# Autodesk Inventor assembly: dribl-2-1
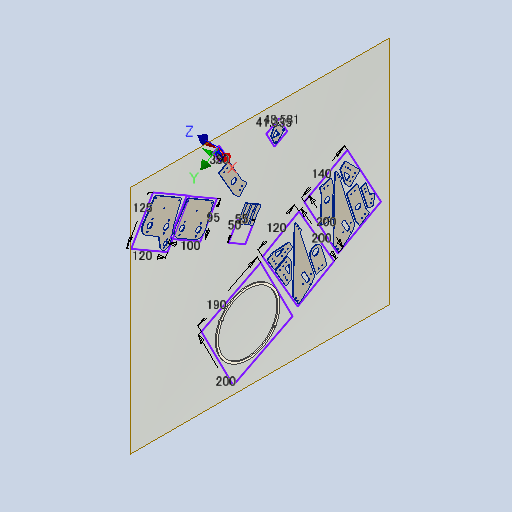
[picture p0: Inventor's stored thumbnail of the model, 512x512]
Saved by Autodesk Inventor 2025.2 (Build 292293000, 293)
## iProperties
Created: 2025-01-15
Part Number: dribl-2-1
Document SubType Name: Assembly
Designer: haruy
Author: haruy
## Documents named in this file (12)
- C:\Users\haruy\Documents\ロボコン\NHK2025\cad\cnc\dribl-2-1.iam
- C:\Users\haruy\Documents\ロボコン\NHK2025\cad\nagahisa\belt_liner\belt_liner_v2_Plate_2.ipt
- C:\Users\haruy\Documents\ロボコン\NHK2025\cad\nagahisa\dribl\dribl-v1-Plate-9.ipt
- C:\Users\haruy\Documents\ロボコン\NHK2025\cad\nagahisa\dribl\dribl-v1-Plate-6.ipt
- C:\Users\haruy\Documents\ロボコン\NHK2025\cad\nagahisa\dribl\dribl-v1-Plate-4.ipt
- C:\Users\haruy\Documents\ロボコン\NHK2025\cad\nagahisa\belt_liner\belt_liner_v2_Plate_20.ipt
- C:\Users\haruy\Documents\ロボコン\NHK2025\cad\nagahisa\dribl\dribl-v1-Plate-8.ipt
- C:\Users\haruy\Documents\ロボコン\NHK2025\cad\nagahisa\belt_liner\belt_liner_v2_Plate_19.ipt
- C:\Users\haruy\Documents\ロボコン\NHK2025\cad\nagahisa\belt_liner\belt_liner_v2_Pom_r.ipt
- C:\Users\haruy\Documents\ロボコン\NHK2025\cad\nagahisa\belt_liner\belt_liner_v4_Plate_2.ipt
- C:\Users\haruy\Documents\ロボコン\NHK2025\cad\nagahisa\belt_liner\belt_liner_v4_Plate_1.ipt
- C:\Users\haruy\Documents\ロボコン\NHK2025\cad\nagahisa\belt_liner\belt_liner_v2_Plate_18.ipt
## Components (19 placed, 11 different names)
1. belt_liner_v2_Plate_2:1 — フラッシュ:1, フラッシュ:4, メイト:6
2. belt_liner_v2_Plate_2:2 — フラッシュ:2, メイト:7, メイト:8, 角度:1
3. dribl-v1-Plate-9:1 — フラッシュ:4, フラッシュ:5, フラッシュ:6, メイト:1
4. dribl-v1-Plate-9:2 — フラッシュ:6, フラッシュ:7, メイト:1
5. dribl-v1-Plate-9:4 — フラッシュ:9, 角度:1
6. dribl-v1-Plate-6:1 — フラッシュ:12, メイト:8
7. dribl-v1-Plate-6:2 — フラッシュ:13, フラッシュ:20, フラッシュ:27, フラッシュ:33
8. dribl-v1-Plate-6:3 — フラッシュ:15, メイト:7, メイト:9
9. dribl-v1-Plate-4:1 — フラッシュ:18, メイト:6
10. belt_liner_v2_Plate_20:1 — メイト:9, フラッシュ:19
11. dribl-v1-Plate-8:1 — フラッシュ:20
12. belt_liner_v2_Plate_19:1 — フラッシュ:21, フラッシュ:22, メイト:10, フラッシュ:24
13. belt_liner_v2_Plate_19:2 — フラッシュ:22, フラッシュ:23, メイト:10, フラッシュ:24, フラッシュ:25, メイト:11
14. belt_liner_v2_Plate_19:3 — フラッシュ:23, フラッシュ:25, メイト:11, フラッシュ:30
15. belt_liner_v2_Pom_r:1 — フラッシュ:26
16. belt_liner_v4_Plate_2:1 — フラッシュ:27, フラッシュ:28, フラッシュ:29, フラッシュ:30
17. belt_liner_v4_Plate_1:1 — フラッシュ:28, フラッシュ:29
18. belt_liner_v2_Plate_18:1 — フラッシュ:31, フラッシュ:32, メイト:12, フラッシュ:33
19. belt_liner_v2_Plate_18:2 — フラッシュ:32, メイト:12
## Relationships (35: Flush 26, Mate 8, Angle 1)
- フラッシュ:1 [Flush]: belt_liner_v2_Plate_2:1
- フラッシュ:2 [Flush]: belt_liner_v2_Plate_2:2
- フラッシュ:4 [Flush]: belt_liner_v2_Plate_2:1 ↔ dribl-v1-Plate-9:1
- フラッシュ:5 [Flush]: dribl-v1-Plate-9:1
- フラッシュ:6 [Flush]: dribl-v1-Plate-9:1 ↔ dribl-v1-Plate-9:2
- フラッシュ:7 [Flush]: dribl-v1-Plate-9:2
- メイト:1 [Mate] (5 mm): dribl-v1-Plate-9:1 ↔ dribl-v1-Plate-9:2
- フラッシュ:9 [Flush]: dribl-v1-Plate-9:4
- フラッシュ:12 [Flush]: dribl-v1-Plate-6:1
- フラッシュ:13 [Flush]: dribl-v1-Plate-6:2
- フラッシュ:15 [Flush]: dribl-v1-Plate-6:3
- フラッシュ:18 [Flush]: dribl-v1-Plate-4:1
- メイト:6 [Mate] (5 mm): belt_liner_v2_Plate_2:1 ↔ dribl-v1-Plate-4:1
- メイト:7 [Mate] (5 mm): belt_liner_v2_Plate_2:2 ↔ dribl-v1-Plate-6:3
- メイト:8 [Mate] (5 mm): belt_liner_v2_Plate_2:2 ↔ dribl-v1-Plate-6:1
- メイト:9 [Mate] (5 mm): dribl-v1-Plate-6:3 ↔ belt_liner_v2_Plate_20:1
- フラッシュ:19 [Flush]: belt_liner_v2_Plate_20:1
- 角度:1 [Angle] (180 deg): belt_liner_v2_Plate_2:2 ↔ dribl-v1-Plate-9:4
- フラッシュ:20 [Flush]: dribl-v1-Plate-6:2 ↔ dribl-v1-Plate-8:1
- フラッシュ:21 [Flush]: belt_liner_v2_Plate_19:1
- フラッシュ:22 [Flush]: belt_liner_v2_Plate_19:1 ↔ belt_liner_v2_Plate_19:2
- フラッシュ:23 [Flush]: belt_liner_v2_Plate_19:2 ↔ belt_liner_v2_Plate_19:3
- メイト:10 [Mate] (5 mm): belt_liner_v2_Plate_19:1 ↔ belt_liner_v2_Plate_19:2
- フラッシュ:24 [Flush]: belt_liner_v2_Plate_19:1 ↔ belt_liner_v2_Plate_19:2
- フラッシュ:25 [Flush]: belt_liner_v2_Plate_19:2 ↔ belt_liner_v2_Plate_19:3
- メイト:11 [Mate] (5 mm): belt_liner_v2_Plate_19:2 ↔ belt_liner_v2_Plate_19:3
- フラッシュ:26 [Flush]: belt_liner_v2_Pom_r:1
- フラッシュ:27 [Flush]: dribl-v1-Plate-6:2 ↔ belt_liner_v4_Plate_2:1
- フラッシュ:28 [Flush]: belt_liner_v4_Plate_2:1 ↔ belt_liner_v4_Plate_1:1
- フラッシュ:29 [Flush]: belt_liner_v4_Plate_2:1 ↔ belt_liner_v4_Plate_1:1
- フラッシュ:30 [Flush]: belt_liner_v2_Plate_19:3 ↔ belt_liner_v4_Plate_2:1
- フラッシュ:31 [Flush]: belt_liner_v2_Plate_18:1
- フラッシュ:32 [Flush]: belt_liner_v2_Plate_18:1 ↔ belt_liner_v2_Plate_18:2
- メイト:12 [Mate] (5 mm): belt_liner_v2_Plate_18:1 ↔ belt_liner_v2_Plate_18:2
- フラッシュ:33 [Flush]: dribl-v1-Plate-6:2 ↔ belt_liner_v2_Plate_18:1
